# Autodesk Inventor assembly: Assembly_Anglerfish_3inch_CompressionCoupling_v0
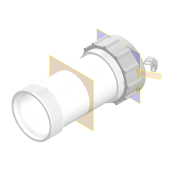
[picture p0: Inventor's stored thumbnail of the model, 180x180]
Saved by Autodesk Inventor 2022 (Build 260153000, 153)
## iProperties
Created: 2022-04-19
Part Number: Assembly_Anglerfish_3inch_CompressionCoupling_v0
Document SubType Name: Assembly
Designer: Prakash Lab
Author: Prakash Lab
## Documents named in this file (7)
- C:\Users\PrakashLab\Documents\Matchboxscope\INVENTOR\Assembly_Anglerfish_3inch_CompressionCoupling_v0.iam
- C:\Users\PrakashLab\Documents\Matchboxscope\INVENTOR\00_Compression_Coupling_3inch_KingBrothers_CPC-3000.ipt
- C:\Users\PrakashLab\Documents\Matchboxscope\INVENTOR\00_Compression_Coupling_3inch_KingBrothers_CPC-3000_rubberring.ipt
- C:\Users\PrakashLab\Documents\Matchboxscope\INVENTOR\00_Compression_Coupling_3inch_KingBrothers_CPC-3000_locking.ipt
- C:\Users\PrakashLab\Documents\Matchboxscope\INVENTOR\00_Powerbank.ipt
- C:\Users\PrakashLab\Documents\Matchboxscope\INVENTOR\Anglerfish_Frontwindow_3inch´_PressureCoupler_V0.ipt
- C:\Users\PrakashLab\Documents\Matchboxscope\INVENTOR\Anglerfish_opticsmodule_v0.iam
## Components (6 placed, 6 different names)
1. 00_Compression_Coupling_3inch_KingBrothers_CPC-3000:1 — Insert:1, Insert:2
2. 00_Compression_Coupling_3inch_KingBrothers_CPC-3000_rubberring:1 — Insert:1, Insert:5
3. 00_Compression_Coupling_3inch_KingBrothers_CPC-3000_locking:1 — Insert:2
4. 00_Powerbank:1
5. Anglerfish_Frontwindow_3inch´_PressureCoupler_V0:1 — Insert:5
6. Anglerfish_opticsmodule_v0:1 [sub-assembly]
## Relationships (7: Insert 4, Mate 3)
- Insert:1: 00_Compression_Coupling_3inch_KingBrothers_CPC-3000:1 ↔ 00_Compression_Coupling_3inch_KingBrothers_CPC-3000_rubberring:1
- Insert:2 (-20 mm): 00_Compression_Coupling_3inch_KingBrothers_CPC-3000:1 ↔ 00_Compression_Coupling_3inch_KingBrothers_CPC-3000_locking:1
- [Mate]: 00_Powerbank:1 ↔ Anglerfish_opticsmodule_v0:1
- [Mate]: 00_Powerbank:1 ↔ Anglerfish_opticsmodule_v0:1
- [Mate] (5 mm): 00_Powerbank:1 ↔ Anglerfish_opticsmodule_v0:1
- Insert:5: 00_Compression_Coupling_3inch_KingBrothers_CPC-3000_rubberring:1 ↔ Anglerfish_Frontwindow_3inch´_PressureCoupler_V0:1
- [Insert]: Anglerfish_Frontwindow_3inch´_PressureCoupler_V0:1 ↔ Anglerfish_opticsmodule_v0:1
## Named parameters: d10_d17 = 0 mm, d11_d18 = 0 mm
